# Autodesk Inventor assembly: Робот_ЕТЗ
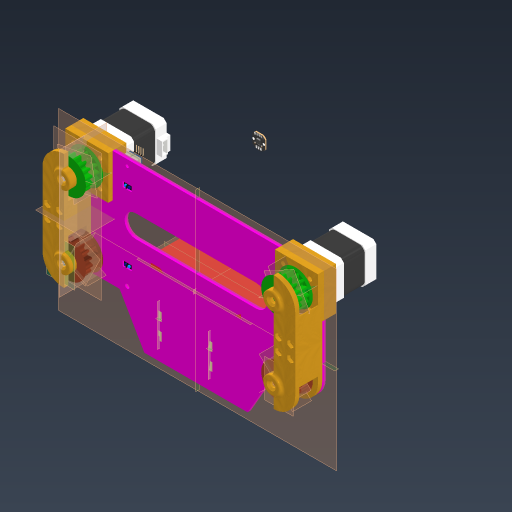
[picture p0: Inventor's stored thumbnail of the model, 512x512]
Saved by Autodesk Inventor 2023.2 (Build 272271030, 271C)
## iProperties
Created: 2025-12-08
Part Number: Робот_ЕТЗ
Document SubType Name: Assembly
Designer: Олег Коноваленко
Author: Олег Коноваленко
## Documents named in this file (15)
- D:\VSOSH_IT_Robotics_ETZ\ETZ\Сonstruction\Робот_ЕТЗ.iam
- D:\VSOSH_IT_Robotics_ETZ\ETZ\Сonstruction\Nema 17.ipt
- D:\VSOSH_IT_Robotics_ETZ\ETZ\Сonstruction\Передняя_крышка.ipt
- D:\VSOSH_IT_Robotics_ETZ\ETZ\Сonstruction\Print\Вал_ведомых_шестерн.ipt
- D:\VSOSH_IT_Robotics_ETZ\ETZ\Сonstruction\Крепление_ведомых_шестерн.ipt
- D:\VSOSH_IT_Robotics_ETZ\ETZ\Сonstruction\Фланцевая_муфта.ipt
- D:\VSOSH_IT_Robotics_ETZ\ETZ\Сonstruction\Вал_ведущих_шестерн.ipt
- D:\VSOSH_IT_Robotics_ETZ\ETZ\Сonstruction\Ведомая_шестерня.ipt
- D:\VSOSH_IT_Robotics_ETZ\ETZ\Сonstruction\Ведущая_шеестерня.ipt
- D:\VSOSH_IT_Robotics_ETZ\ETZ\Сonstruction\Крепление_ведомых_шестерн_MIR1.ipt
- D:\VSOSH_IT_Robotics_ETZ\ETZ\Сonstruction\TCRT5000.ipt
- D:\VSOSH_IT_Robotics_ETZ\ETZ\Сonstruction\Крепление_TCRT.ipt
- D:\VSOSH_IT_Robotics_ETZ\ETZ\Сonstruction\AS5048A Magnetic Encoder - B.ipt
- D:\VSOSH_IT_Robotics_ETZ\ETZ\Сonstruction\Выступ_под_крепление_маркера.ipt
- D:\VSOSH_IT_Robotics_ETZ\ETZ\Сonstruction\Рёбра_жёсткости.ipt
## Components (21 placed, 14 different names)
1. Nema 17:1 — Совмещение:78, Заподлицо:26, Угол:1
2. Передняя_крышка:1 — Заподлицо:27, Совмещение:79, Совмещение:80, Совмещение:81, Заподлицо:28, Совмещение:82, Заподлицо:35, Совмещение:95, Совмещение:96, Заподлицо:36, Совмещение:98, Совмещение:99, Заподлицо:38, Совмещение:100, Совмещение:101
3. Вал_ведомых_шестерн:1 — Заподлицо:21, Совмещение:76, Совмещение:85
4. Крепление_ведомых_шестерн:1 — Заподлицо:21, Совмещение:64, Совмещение:68, Совмещение:70, Заподлицо:23, Совмещение:73, Совмещение:75, Совмещение:76, Заподлицо:27, Совмещение:79, Совмещение:80, Угол:1, Совмещение:97
5. Фланцевая_муфта:1 — Совмещение:64, Совмещение:65, Совмещение:68, Совмещение:74, Совмещение:78, Заподлицо:26
6. Вал_ведущих_шестерн:1 — Совмещение:70, Заподлицо:23
7. Ведомая_шестерня:1 — Совмещение:75, Совмещение:85
8. Ведущая_шестерня:2 — Совмещение:65, Совмещение:73, Совмещение:74
9. Крепление_ведомых_шестерн_MIR1:1 — Совмещение:81, Заподлицо:28, Совмещение:82, Совмещение:83, Совмещение:84, Совмещение:86, Совмещение:87, Угол:2
10. Ведущая_шестерня:3 — Совмещение:86, Совмещение:87, Совмещение:88, Совмещение:89, Совмещение:91
11. Ведомая_шестерня:2 — Совмещение:83, Совмещение:84
12. Nema 17:2 — Совмещение:90, Заподлицо:29, Угол:2
13. Фланцевая_муфта:2 — Совмещение:88, Совмещение:89, Совмещение:90, Заподлицо:29, Совмещение:91
14. TCRT5000:1 — Совмещение:92, Заподлицо:30, Заподлицо:31
15. Крепление_TCRT:1 — Совмещение:92, Заподлицо:30, Заподлицо:31, Совмещение:95, Заподлицо:36, Заподлицо:37
16. TCRT5000:2
17. Крепление_TCRT:2 — Заподлицо:35, Совмещение:96, Заподлицо:37, Совмещение:97
18. AS5048A Magnetic Encoder - B:1
19. Выступ_под_крепление_маркера:1 — Совмещение:98, Совмещение:99, Заподлицо:38
20. Рёбра_жёсткости:1 — Совмещение:101
21. Рёбра_жёсткости:2 — Совмещение:100
## Relationships (47: Mate 31, Flush 14, Angle 2)
- Заподлицо:21 [Flush]: Вал_ведомых_шестерн:1 ↔ Крепление_ведомых_шестерн:1
- Совмещение:64 [Mate]: Крепление_ведомых_шестерн:1 ↔ Фланцевая_муфта:1
- Совмещение:65 [Mate]: Фланцевая_муфта:1 ↔ Ведущая_шестерня:2
- Совмещение:68 [Mate]: Крепление_ведомых_шестерн:1 ↔ Фланцевая_муфта:1
- Совмещение:70 [Mate]: Крепление_ведомых_шестерн:1 ↔ Вал_ведущих_шестерн:1
- Заподлицо:23 [Flush]: Крепление_ведомых_шестерн:1 ↔ Вал_ведущих_шестерн:1
- Совмещение:73 [Mate] (0.5 mm): Крепление_ведомых_шестерн:1 ↔ Ведущая_шестерня:2
- Совмещение:74 [Mate]: Фланцевая_муфта:1 ↔ Ведущая_шестерня:2
- Совмещение:75 [Mate] (0.5 mm): Крепление_ведомых_шестерн:1 ↔ Ведомая_шестерня:1
- Совмещение:76 [Mate]: Вал_ведомых_шестерн:1 ↔ Крепление_ведомых_шестерн:1
- Совмещение:78 [Mate]: Nema 17:1 ↔ Фланцевая_муфта:1
- Заподлицо:26 [Flush]: Nema 17:1 ↔ Фланцевая_муфта:1
- Заподлицо:27 [Flush]: Передняя_крышка:1 ↔ Крепление_ведомых_шестерн:1
- Совмещение:79 [Mate]: Передняя_крышка:1 ↔ Крепление_ведомых_шестерн:1
- Совмещение:80 [Mate]: Передняя_крышка:1 ↔ Крепление_ведомых_шестерн:1
- Совмещение:81 [Mate]: Передняя_крышка:1 ↔ Крепление_ведомых_шестерн_MIR1:1
- Заподлицо:28 [Flush]: Передняя_крышка:1 ↔ Крепление_ведомых_шестерн_MIR1:1
- Совмещение:82 [Mate]: Передняя_крышка:1 ↔ Крепление_ведомых_шестерн_MIR1:1
- Совмещение:83 [Mate] (0.5 mm): Крепление_ведомых_шестерн_MIR1:1 ↔ Ведомая_шестерня:2
- Совмещение:84 [Mate]: Крепление_ведомых_шестерн_MIR1:1 ↔ Ведомая_шестерня:2
- Совмещение:85 [Mate]: Вал_ведомых_шестерн:1 ↔ Ведомая_шестерня:1
- Совмещение:86 [Mate] (0.5 mm): Крепление_ведомых_шестерн_MIR1:1 ↔ Ведущая_шестерня:3
- Совмещение:87 [Mate]: Крепление_ведомых_шестерн_MIR1:1 ↔ Ведущая_шестерня:3
- Угол:1 [Angle] (0 deg): Nema 17:1 ↔ Крепление_ведомых_шестерн:1
- Совмещение:88 [Mate]: Ведущая_шестерня:3 ↔ Фланцевая_муфта:2
- Совмещение:89 [Mate]: Ведущая_шестерня:3 ↔ Фланцевая_муфта:2
- Совмещение:90 [Mate]: Nema 17:2 ↔ Фланцевая_муфта:2
- Заподлицо:29 [Flush]: Nema 17:2 ↔ Фланцевая_муфта:2
- Совмещение:91 [Mate]: Ведущая_шестерня:3 ↔ Фланцевая_муфта:2
- Угол:2 [Angle] (0 deg): Крепление_ведомых_шестерн_MIR1:1 ↔ Nema 17:2
- Совмещение:92 [Mate]: TCRT5000:1 ↔ Крепление_TCRT:1
- Заподлицо:30 [Flush]: TCRT5000:1 ↔ Крепление_TCRT:1
- Заподлицо:31 [Flush]: TCRT5000:1 ↔ Крепление_TCRT:1
- [Mate]: TCRT5000:2 ↔ Крепление_TCRT:2
- [Flush]: TCRT5000:2 ↔ Крепление_TCRT:2
- [Flush]: TCRT5000:2 ↔ Крепление_TCRT:2
- Заподлицо:35 [Flush]: Передняя_крышка:1 ↔ Крепление_TCRT:2
- Совмещение:95 [Mate]: Передняя_крышка:1 ↔ Крепление_TCRT:1
- Совмещение:96 [Mate]: Передняя_крышка:1 ↔ Крепление_TCRT:2
- Заподлицо:36 [Flush]: Передняя_крышка:1 ↔ Крепление_TCRT:1
- Заподлицо:37 [Flush]: Крепление_TCRT:1 ↔ Крепление_TCRT:2
- Совмещение:97 [Mate] (10 mm): Крепление_ведомых_шестерн:1 ↔ Крепление_TCRT:2
- Совмещение:98 [Mate]: Передняя_крышка:1 ↔ Выступ_под_крепление_маркера:1
- Совмещение:99 [Mate]: Передняя_крышка:1 ↔ Выступ_под_крепление_маркера:1
- Заподлицо:38 [Flush] (15 mm): Передняя_крышка:1 ↔ Выступ_под_крепление_маркера:1
- Совмещение:100 [Mate]: Передняя_крышка:1 ↔ Рёбра_жёсткости:2
- Совмещение:101 [Mate]: Передняя_крышка:1 ↔ Рёбра_жёсткости:1
## Named parameters: d165_d160 = 0 mm, d166_d161 = 0 mm, d167_d162 = 0 mm
